# Autodesk Inventor assembly: アームアセンブリ2
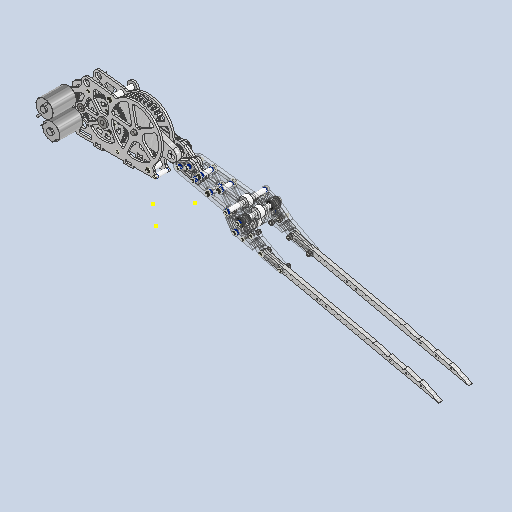
[picture p0: Inventor's stored thumbnail of the model, 512x512]
Saved by Autodesk Inventor 2023.1 (Build 271208000, 208)
## iProperties
Created: 2022-06-19
Part Number: アームアセンブリ2
Document SubType Name: Assembly
Designer: muzho
Mass: 875.353 g
Surface Area: 2137.13 cm^2
Volume: 305.154 cm^3
Density: 2.86856 g/cm^3
Author: muzho
## Documents named in this file (37)
- C:\Users\muzho\Documents\srdc\srdc_2\アーム\アームアセンブリ.iam
- C:\Users\muzho\Documents\srdc\srdc_2\アーム\主フレーム.ipt
- C:\Users\muzho\Documents\srdc\srdc_2\アーム\右フレーム.ipt
- C:\Users\muzho\Documents\srdc\srdc_2\アーム(世古)\既製品\スペーサーm3-16　簡易筒型.ipt
- C:\Users\muzho\Documents\srdc\srdc_2\アーム\左フレーム.ipt
- C:\Users\muzho\Documents\srdc\srdc_2\アーム\ギア\最終段m2z40.ipt
- C:\Users\muzho\Documents\srdc\srdc_2\アーム(世古)\アーム 駆動フリー節.ipt
- C:\Users\muzho\Documents\srdc\srdc_2\スペーサ\l5.ipt
- C:\Users\muzho\Documents\srdc\srdc_2\ワッシャー\チタンワッシャー　4.2-10-1.ipt
- C:\Users\muzho\Documents\srdc\srdc_2\ドライメット\w3f6-8a.ipt
- C:\Users\muzho\Documents\srdc\srdc_2\アーム(世古)\アーム 小さいカム押さえるやつ.ipt
- C:\Users\muzho\Documents\srdc\srdc_2\ねじ\M3ボタンボルト25.ipt
- C:\Users\muzho\Documents\srdc\srdc_2\アーム(世古)\アーム 小さいカム.ipt
- C:\Users\muzho\Documents\srdc\srdc_2\アーム(世古)\アーム 中間節.ipt
- C:\Users\muzho\Documents\srdc\srdc_2\アーム(世古)\アーム 中間節(ミラー).ipt
- C:\Users\muzho\Documents\srdc\srdc_2\スペーサ\l14.ipt
- C:\Users\muzho\Documents\srdc\srdc_2\アーム(世古)\アーム 揺動節.ipt
- C:\Users\muzho\Documents\srdc\srdc_2\ピン\φ6l25.ipt
- C:\Users\muzho\Documents\srdc\srdc_2\ドライメット\w6f14-16.ipt
- C:\Users\muzho\Documents\srdc\srdc_2\ねじ\SB　10mmなべネジ.ipt
- C:\Users\muzho\Documents\srdc\srdc_2\ねじ\SB　6mm皿ネジ.ipt
- C:\Users\muzho\Documents\srdc\srdc_2\ねじ\ナイロンナットm3.ipt
- C:\Users\muzho\Documents\srdc\srdc_2\ピン\φ6l30.ipt
- C:\Users\muzho\Documents\srdc\srdc_2\ベアリング\φ6φ15a.ipt
- C:\Users\muzho\Documents\srdc\srdc_2\アーム\ギア\二段_多段ギア.iam
- C:\Users\muzho\Documents\srdc\srdc_2\アーム\ギア\初段_多段ギア.iam
- C:\Users\muzho\Documents\srdc\srdc_2\ベアリング\Φ4-9a.ipt
- C:\Users\muzho\Documents\srdc\srdc_2\ピン\φ4l25.ipt
- C:\Users\muzho\Documents\srdc\srdc_2\モータ\M-RS-380.ipt
- C:\Users\muzho\Documents\srdc\srdc_2\ねじ\M2.6 ボルト 6mm.ipt
- C:\Users\muzho\Documents\srdc\srdc_2\スペーサ\m4l35.ipt
- C:\Users\muzho\Documents\srdc\srdc_2\ねじ\SB　M4 8mm なべネジ.ipt
- C:\Users\muzho\Documents\srdc\srdc_2\ねじ\SB　6mmなべネジ.ipt
- C:\Users\muzho\Documents\srdc\srdc_2\アーム(世古)\アーム 中間節 中詰め.ipt
- C:\Users\muzho\Documents\srdc\srdc_2\アーム(世古)\アーム ツインロッドアーム先端アセンブリ.iam
- C:\Users\muzho\Documents\srdc\srdc_2\ねじ\SB　8mmなべネジ.ipt
- C:\Users\muzho\Documents\srdc\srdc_2\スペーサ\l16.ipt
## Components (77 placed, 36 different names)
1. 主フレーム:1 — メイト:1, メイト:3, メイト:4, 挿入:19, 挿入:20, 挿入:23, 挿入:26, 挿入:46, メイト:24, 挿入:47, メイト:26, 挿入:49, 挿入:50, 挿入:51, 挿入:57, 挿入:58, 挿入:75, 挿入:77, 挿入:78, 挿入:95, 挿入:96, 挿入:98
2. 右フレーム:1 — メイト:1, 挿入:1, メイト:5, 挿入:25, 挿入:37, メイト:25, 挿入:48, 挿入:52, 挿入:53, メイト:27, 挿入:54, 挿入:55, 挿入:56, 挿入:60, 挿入:74, 挿入:76, メイト:33, 挿入:83, 挿入:97
3. スペーサーm3-16　簡易筒型:1 — 挿入:1, 挿入:19
4. 左フレーム:1 — メイト:3, メイト:4, メイト:6, 挿入:5, 挿入:59, 挿入:64, 挿入:73, 挿入:81, 挿入:84
5. 最終段m2z40:1 — メイト:5, メイト:7, メイト:8, メイト:9, 挿入:6, 挿入:7, 挿入:8, 挿入:9, 挿入:27, メイト:21
6. アーム 駆動フリー節:1 — メイト:6, メイト:7, 挿入:12, 挿入:16, メイト:15, 挿入:34, 挿入:35, 挿入:36
7. l5:1 — 挿入:16, 挿入:28
8. チタンワッシャー　4.2-10-1:1 — 挿入:28, 挿入:29
9. w3f6-8a:1 — 挿入:5
10. アーム 小さいカム押さえるやつ:1 — メイト:8, メイト:9, 挿入:6, 挿入:10
11. M3ボタンボルト25:1 — 挿入:7, メイト:10
12. M3ボタンボルト25:2 — 挿入:8, メイト:11
13. M3ボタンボルト25:3 — 挿入:9
14. アーム 小さいカム:1 — メイト:10, メイト:11, 挿入:10, 挿入:12, 挿入:33
15. アーム 中間節:1 — メイト:16, メイト:17, 挿入:22, 挿入:30, メイト:30, 挿入:79
16. l14:1 — 挿入:20, メイト:13
17. アーム 揺動節:1 — メイト:13, メイト:14, 挿入:30, 挿入:99
18. アーム 中間節(ミラー):2 — メイト:14, メイト:15, メイト:16, メイト:17, 挿入:22, 挿入:24, 挿入:31, 挿入:32
19. φ6l25:1 — 挿入:23
20. w6f14-16:1 — 挿入:24, 挿入:33
21. w3f6-8a:2 — 挿入:25
22. w3f6-8a:3 — 挿入:26, 挿入:27
23. SB　10mmなべネジ:1 — 挿入:29
24. SB　6mm皿ネジ:1 — 挿入:32
25. SB　6mm皿ネジ:2 — 挿入:31
26. ナイロンナットm3:1 — 挿入:36, メイト:19
27. ナイロンナットm3:2 — 挿入:34, メイト:18, メイト:19
28. ナイロンナットm3:3 — 挿入:35, メイト:18
29. φ6l30:1 — 挿入:39, メイト:20
30. φ6φ15a:1 — 挿入:95
31. φ6φ15a:2 — 挿入:37, 挿入:39
32. 二段_多段ギア:1 [sub-assembly] — メイト:20, メイト:21
33. Φ4-9a:1 — 挿入:46
34. Φ4-9a:2 — 挿入:45, メイト:33, 挿入:83, 挿入:94
35. φ4l25:1 — 挿入:45, メイト:37
36. M-RS-380:1 — メイト:26, 挿入:49
37. M-RS-380:2 — メイト:25, 挿入:48
38. M-RS-380:3 — メイト:27, 挿入:54
39. M-RS-380:4 — メイト:24, 挿入:47
40. M2.6 ボルト 6mm:1 — 挿入:56
41. M2.6 ボルト 6mm:2 — 挿入:55
42. M2.6 ボルト 6mm:3 — 挿入:53
43. M2.6 ボルト 6mm:4 — 挿入:57
44. M2.6 ボルト 6mm:5 — 挿入:51
45. M2.6 ボルト 6mm:6 — 挿入:50
46. M2.6 ボルト 6mm:7 — 挿入:58
47. M2.6 ボルト 6mm:9 — 挿入:52
48. m4l35:1 — 挿入:59, 挿入:60
49. m4l35:2 — 挿入:64
50. SB　M4 8mm なべネジ:1
51. SB　6mmなべネジ:1
52. SB　6mmなべネジ:2
53. SB　6mmなべネジ:4 — 挿入:75
54. SB　M4 8mm なべネジ:2 — 挿入:73
55. SB　M4 8mm なべネジ:3 — 挿入:74
56. SB　6mmなべネジ:5 — 挿入:76
57. SB　6mmなべネジ:6 — 挿入:77
58. SB　6mmなべネジ:7 — 挿入:78
59. 初段_多段ギア:1 [sub-assembly] — メイト:37, 挿入:94
60. アーム 中間節 中詰め:1 — メイト:30, 挿入:79, メイト:31, 挿入:80
61. アーム 中間節 中詰め:2 — メイト:31, 挿入:80, メイト:34, メイト:35, メイト:36
62. SB　M4 8mm なべネジ:4 — 挿入:81
63. アーム ツインロッドアーム先端アセンブリ:1 [sub-assembly] — 挿入:85, 挿入:86, 挿入:87, メイト:36, 挿入:88, 挿入:89, 挿入:90, 挿入:91, 挿入:92, 挿入:93
64. SB　6mmなべネジ:8 — 挿入:84
65. SB　8mmなべネジ:1 — 挿入:88
66. SB　8mmなべネジ:2 — 挿入:89
67. SB　8mmなべネジ:3 — 挿入:90
68. l16:1 — 挿入:85, メイト:35
69. l16:2 — 挿入:86, メイト:34
70. l16:3 — 挿入:87
71. SB　8mmなべネジ:4 — 挿入:92
72. SB　8mmなべネジ:5 — 挿入:91
73. SB　8mmなべネジ:6 — 挿入:93
74. l16:4 — 挿入:96
75. l16:5 — 挿入:97
76. l16:6 — 挿入:98
77. w3f6-8a:4 — 挿入:99
## Relationships (101: Insert 71, Mate 30)
- メイト:1 [Mate]: 主フレーム:1 ↔ 右フレーム:1
- 挿入:1 [Insert]: 右フレーム:1 ↔ スペーサーm3-16　簡易筒型:1
- メイト:3 [Mate]: 主フレーム:1 ↔ 左フレーム:1
- メイト:4 [Mate]: 主フレーム:1 ↔ 左フレーム:1
- メイト:5 [Mate]: 右フレーム:1 ↔ 最終段m2z40:1
- メイト:6 [Mate]: 左フレーム:1 ↔ アーム 駆動フリー節:1
- 挿入:5 [Insert]: 左フレーム:1 ↔ w3f6-8a:1
- メイト:7 [Mate]: 最終段m2z40:1 ↔ アーム 駆動フリー節:1
- メイト:8 [Mate]: 最終段m2z40:1 ↔ アーム 小さいカム押さえるやつ:1
- メイト:9 [Mate]: 最終段m2z40:1 ↔ アーム 小さいカム押さえるやつ:1
- 挿入:6 [Insert]: 最終段m2z40:1 ↔ アーム 小さいカム押さえるやつ:1
- 挿入:7 [Insert]: 最終段m2z40:1 ↔ M3ボタンボルト25:1
- 挿入:8 [Insert]: 最終段m2z40:1 ↔ M3ボタンボルト25:2
- 挿入:9 [Insert]: 最終段m2z40:1 ↔ M3ボタンボルト25:3
- メイト:10 [Mate]: M3ボタンボルト25:1 ↔ アーム 小さいカム:1
- メイト:11 [Mate]: M3ボタンボルト25:2 ↔ アーム 小さいカム:1
- 挿入:10 [Insert]: アーム 小さいカム押さえるやつ:1 ↔ アーム 小さいカム:1
- 挿入:12 [Insert]: アーム 駆動フリー節:1 ↔ アーム 小さいカム:1
- 挿入:16 [Insert]: アーム 駆動フリー節:1 ↔ l5:1
- 挿入:19 [Insert]: 主フレーム:1 ↔ スペーサーm3-16　簡易筒型:1
- 挿入:20 [Insert]: 主フレーム:1 ↔ l14:1
- メイト:13 [Mate]: l14:1 ↔ アーム 揺動節:1
- メイト:14 [Mate]: アーム 揺動節:1 ↔ アーム 中間節(ミラー):2
- メイト:15 [Mate]: アーム 駆動フリー節:1 ↔ アーム 中間節(ミラー):2
- メイト:16 [Mate]: アーム 中間節:1 ↔ アーム 中間節(ミラー):2
- メイト:17 [Mate]: アーム 中間節:1 ↔ アーム 中間節(ミラー):2
- 挿入:22 [Insert]: アーム 中間節:1 ↔ アーム 中間節(ミラー):2
- 挿入:23 [Insert]: 主フレーム:1 ↔ φ6l25:1
- 挿入:24 [Insert]: アーム 中間節(ミラー):2 ↔ w6f14-16:1
- 挿入:25 [Insert]: 右フレーム:1 ↔ w3f6-8a:2
- 挿入:26 [Insert]: 主フレーム:1 ↔ w3f6-8a:3
- 挿入:27 [Insert] (0.6 mm): 最終段m2z40:1 ↔ w3f6-8a:3
- 挿入:28 [Insert]: l5:1 ↔ チタンワッシャー　4.2-10-1:1
- 挿入:29 [Insert]: チタンワッシャー　4.2-10-1:1 ↔ SB　10mmなべネジ:1
- 挿入:30 [Insert] (0.25 mm): アーム 中間節:1 ↔ アーム 揺動節:1
- 挿入:31 [Insert]: アーム 中間節(ミラー):2 ↔ SB　6mm皿ネジ:2
- 挿入:32 [Insert]: アーム 中間節(ミラー):2 ↔ SB　6mm皿ネジ:1
- 挿入:33 [Insert] (0.5 mm): アーム 小さいカム:1 ↔ w6f14-16:1
- 挿入:34 [Insert]: アーム 駆動フリー節:1 ↔ ナイロンナットm3:2
- 挿入:35 [Insert]: アーム 駆動フリー節:1 ↔ ナイロンナットm3:3
- 挿入:36 [Insert]: アーム 駆動フリー節:1 ↔ ナイロンナットm3:1
- メイト:18 [Mate]: ナイロンナットm3:2 ↔ ナイロンナットm3:3
- メイト:19 [Mate]: ナイロンナットm3:1 ↔ ナイロンナットm3:2
- 挿入:37 [Insert]: 右フレーム:1 ↔ φ6φ15a:2
- 挿入:39 [Insert]: φ6l30:1 ↔ φ6φ15a:2
- メイト:20 [Mate]: φ6l30:1 ↔ 二段_多段ギア:1
- メイト:21 [Mate] (0.5 mm): 最終段m2z40:1 ↔ 二段_多段ギア:1
- 挿入:45 [Insert]: Φ4-9a:2 ↔ φ4l25:1
- 挿入:46 [Insert]: 主フレーム:1 ↔ Φ4-9a:1
- メイト:24 [Mate]: 主フレーム:1 ↔ M-RS-380:4
- 挿入:47 [Insert]: 主フレーム:1 ↔ M-RS-380:4
- メイト:25 [Mate]: 右フレーム:1 ↔ M-RS-380:2
- 挿入:48 [Insert]: 右フレーム:1 ↔ M-RS-380:2
- メイト:26 [Mate]: 主フレーム:1 ↔ M-RS-380:1
- 挿入:49 [Insert]: 主フレーム:1 ↔ M-RS-380:1
- 挿入:50 [Insert]: 主フレーム:1 ↔ M2.6 ボルト 6mm:6
- 挿入:51 [Insert]: 主フレーム:1 ↔ M2.6 ボルト 6mm:5
- 挿入:52 [Insert]: 右フレーム:1 ↔ M2.6 ボルト 6mm:9
- 挿入:53 [Insert]: 右フレーム:1 ↔ M2.6 ボルト 6mm:3
- メイト:27 [Mate]: 右フレーム:1 ↔ M-RS-380:3
- 挿入:54 [Insert]: 右フレーム:1 ↔ M-RS-380:3
- 挿入:55 [Insert]: 右フレーム:1 ↔ M2.6 ボルト 6mm:2
- 挿入:56 [Insert]: 右フレーム:1 ↔ M2.6 ボルト 6mm:1
- 挿入:57 [Insert]: 主フレーム:1 ↔ M2.6 ボルト 6mm:4
- 挿入:58 [Insert]: 主フレーム:1 ↔ M2.6 ボルト 6mm:7
- 挿入:59 [Insert]: 左フレーム:1 ↔ m4l35:1
- 挿入:60 [Insert]: 右フレーム:1 ↔ m4l35:1
- 挿入:64 [Insert]: 左フレーム:1 ↔ m4l35:2
- 挿入:73 [Insert]: 左フレーム:1 ↔ SB　M4 8mm なべネジ:2
- 挿入:74 [Insert]: 右フレーム:1 ↔ SB　M4 8mm なべネジ:3
- 挿入:75 [Insert]: 主フレーム:1 ↔ SB　6mmなべネジ:4
- 挿入:76 [Insert]: 右フレーム:1 ↔ SB　6mmなべネジ:5
- 挿入:77 [Insert]: 主フレーム:1 ↔ SB　6mmなべネジ:6
- 挿入:78 [Insert]: 主フレーム:1 ↔ SB　6mmなべネジ:7
- メイト:30 [Mate]: アーム 中間節:1 ↔ アーム 中間節 中詰め:1
- 挿入:79 [Insert]: アーム 中間節:1 ↔ アーム 中間節 中詰め:1
- メイト:31 [Mate]: アーム 中間節 中詰め:1 ↔ アーム 中間節 中詰め:2
- 挿入:80 [Insert]: アーム 中間節 中詰め:1 ↔ アーム 中間節 中詰め:2
- 挿入:81 [Insert]: 左フレーム:1 ↔ SB　M4 8mm なべネジ:4
- メイト:33 [Mate]: 右フレーム:1 ↔ Φ4-9a:2
- 挿入:83 [Insert]: 右フレーム:1 ↔ Φ4-9a:2
- 挿入:84 [Insert]: 左フレーム:1 ↔ SB　6mmなべネジ:8
- 挿入:85 [Insert]: アーム ツインロッドアーム先端アセンブリ:1 ↔ l16:1
- 挿入:86 [Insert]: アーム ツインロッドアーム先端アセンブリ:1 ↔ l16:2
- 挿入:87 [Insert]: アーム ツインロッドアーム先端アセンブリ:1 ↔ l16:3
- メイト:34 [Mate]: アーム 中間節 中詰め:2 ↔ l16:2
- メイト:35 [Mate]: アーム 中間節 中詰め:2 ↔ l16:1
- メイト:36 [Mate]: アーム 中間節 中詰め:2 ↔ アーム ツインロッドアーム先端アセンブリ:1
- 挿入:88 [Insert]: アーム ツインロッドアーム先端アセンブリ:1 ↔ SB　8mmなべネジ:1
- 挿入:89 [Insert]: アーム ツインロッドアーム先端アセンブリ:1 ↔ SB　8mmなべネジ:2
- 挿入:90 [Insert]: アーム ツインロッドアーム先端アセンブリ:1 ↔ SB　8mmなべネジ:3
- 挿入:91 [Insert]: アーム ツインロッドアーム先端アセンブリ:1 ↔ SB　8mmなべネジ:5
- 挿入:92 [Insert]: アーム ツインロッドアーム先端アセンブリ:1 ↔ SB　8mmなべネジ:4
- 挿入:93 [Insert]: アーム ツインロッドアーム先端アセンブリ:1 ↔ SB　8mmなべネジ:6
- メイト:37 [Mate]: φ4l25:1 ↔ 初段_多段ギア:1
- 挿入:94 [Insert] (0.6 mm): Φ4-9a:2 ↔ 初段_多段ギア:1
- 挿入:95 [Insert]: 主フレーム:1 ↔ φ6φ15a:1
- 挿入:96 [Insert]: 主フレーム:1 ↔ l16:4
- 挿入:97 [Insert]: 右フレーム:1 ↔ l16:5
- 挿入:98 [Insert]: 主フレーム:1 ↔ l16:6
- 挿入:99 [Insert]: アーム 揺動節:1 ↔ w3f6-8a:4
